# Autodesk Inventor assembly: wheel_screw_joint
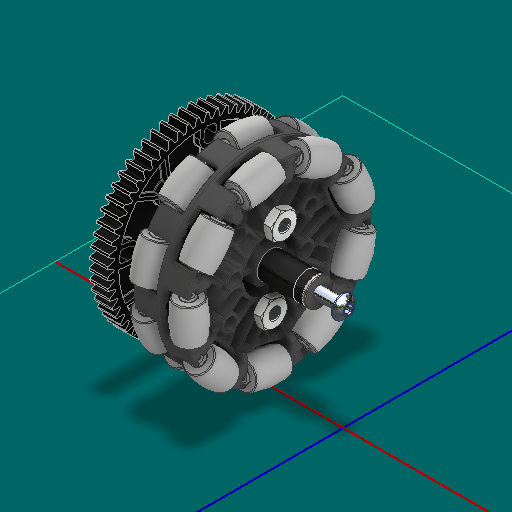
[picture p0: Inventor's stored thumbnail of the model, 512x512]
Saved by Autodesk Inventor 2025 (Build 290162000, 162)
## iProperties
Created: 2024-08-16
Part Number: wheel_screw_joint
Document SubType Name: Assembly
Designer: averey
Author: averey
## Documents named in this file (17)
- C:\Users\avere\vex_robotics_high_stakes\hardware\cad\ATLAS\chassis\drive_pod\wheel_screw_joint.iam
- C:\Users\avere\vex_robotics_high_stakes\hardware\cad\VEX-CAD-Inventor\Structure\Hardware\Screw Steel - Star\SScrew Star Smooth 2.500.ipt
- C:\Users\avere\vex_robotics_high_stakes\hardware\cad\VEX-CAD-Inventor\Structure\Hardware\Screw Steel - Star.ipt
- C:\Users\avere\vex_robotics_high_stakes\hardware\cad\VEX-CAD-Inventor\Motion\Wheels\Omni Wheel\2.75 Omni AS, No Insert.iam
- C:\Users\avere\vex_robotics_high_stakes\hardware\cad\VEX-CAD-Inventor\Motion\Wheels\Omni Wheel.iam
- C:\Users\avere\vex_robotics_high_stakes\hardware\cad\custom_parts\modified_parts\Half Cut HS 60T Gear.ipt
- C:\Users\avere\vex_robotics_high_stakes\hardware\cad\VEX-CAD-Inventor\Motion\Spacers\Spacer Nylon .375 OD\NSpacer .375 OD x .375.ipt
- C:\Users\avere\vex_robotics_high_stakes\hardware\cad\VEX-CAD-Inventor\Motion\Spacers\Spacer Nylon .375 OD.ipt
- C:\Users\avere\vex_robotics_high_stakes\hardware\cad\VEX-CAD-Inventor\Motion\Spacers\Washer Steel\SWasher .375 OD x .015625.ipt
- C:\Users\avere\vex_robotics_high_stakes\hardware\cad\VEX-CAD-Inventor\Motion\Spacers\Washer Steel.ipt
- C:\Users\avere\vex_robotics_high_stakes\hardware\cad\VEX-CAD-Inventor\Motion\Spacers\Washer Steel\SWasher .375 OD x .031250.ipt
- C:\Users\avere\vex_robotics_high_stakes\hardware\cad\VEX-CAD-Inventor\Motion\Spacers\Washer Steel\SWasher .375 OD x .062500.ipt
- C:\Users\avere\vex_robotics_high_stakes\hardware\cad\VEX-CAD-Inventor\Structure\Hardware\Screw Steel - Star\SScrew Star Smooth 1.500.ipt
- C:\Users\avere\vex_robotics_high_stakes\hardware\cad\VEX-CAD-Inventor\Structure\Hardware\Nut Nylon\Nut Nylon - White.ipt
- C:\Users\avere\vex_robotics_high_stakes\hardware\cad\VEX-CAD-Inventor\Structure\Hardware\Nut Nylon.ipt
- C:\Users\avere\vex_robotics_high_stakes\hardware\cad\VEX-CAD-Inventor\Motion\Spacers\Spacer Nylon .375 OD\NSpacer .375 OD x .125.ipt
- C:\Users\avere\vex_robotics_high_stakes\hardware\cad\VEX-CAD-Inventor\Motion\Spacers\Spacer Nylon .375 OD\NSpacer .375 OD x .500.ipt
## Components (19 placed, 11 different names)
1. SScrew Star Smooth 2.500:1 — Mate:1, Mate:2
2. 2.75 Omni AS, No Insert:1 [sub-assembly] — Insert:9, Insert:10, Insert:11, Insert:12, Insert:18
3. Half Cut HS 60T Gear:1 — Mate:3, Insert:13, Insert:14
4. NSpacer .375 OD x .375:1 — Insert:5, Insert:9
5. SWasher .375 OD x .015625:1 — Insert:4
6. SWasher .375 OD x .031250:2 — Insert:3, Insert:4, Mate:3
7. SWasher .375 OD x .062500:3 — Insert:3, Insert:5
8. NSpacer .375 OD x .375:2 — Insert:10
9. SWasher .375 OD x .015625:4
10. SWasher .375 OD x .031250:5
11. SWasher .375 OD x .062500:6
12. SScrew Star Smooth 1.500:2 — Insert:14
13. SScrew Star Smooth 1.500:3 — Insert:13
14. Nut Nylon - White:1 — Insert:11
15. Nut Nylon - White:2 — Insert:12
16. NSpacer .375 OD x .125:3 — Insert:16, Insert:17
17. NSpacer .375 OD x .500:4 — Insert:16, Insert:18
18. SWasher .375 OD x .015625:7 — Insert:15
19. SWasher .375 OD x .031250:8 — Insert:15, Insert:17
## Relationships (21: Insert 18, Mate 3)
- [Insert] (25.4 mm): SScrew Star Smooth 2.500:1 ↔ 2.75 Omni AS, No Insert:1
- [Insert] (9.1281 mm): 2.75 Omni AS, No Insert:1 ↔ Half Cut HS 60T Gear:1
- Mate:1: SScrew Star Smooth 2.500:1
- Mate:2: SScrew Star Smooth 2.500:1
- Insert:3: SWasher .375 OD x .031250:2 ↔ SWasher .375 OD x .062500:3
- Insert:4: SWasher .375 OD x .015625:1 ↔ SWasher .375 OD x .031250:2
- Insert:5: NSpacer .375 OD x .375:1 ↔ SWasher .375 OD x .062500:3
- [Insert]: SWasher .375 OD x .031250:5 ↔ SWasher .375 OD x .062500:6
- [Insert]: SWasher .375 OD x .015625:4 ↔ SWasher .375 OD x .031250:5
- [Insert]: NSpacer .375 OD x .375:2 ↔ SWasher .375 OD x .062500:6
- Insert:9: 2.75 Omni AS, No Insert:1 ↔ NSpacer .375 OD x .375:1
- Insert:10: 2.75 Omni AS, No Insert:1 ↔ NSpacer .375 OD x .375:2
- Mate:3: Half Cut HS 60T Gear:1 ↔ SWasher .375 OD x .031250:2
- Insert:11: 2.75 Omni AS, No Insert:1 ↔ Nut Nylon - White:1
- Insert:12: 2.75 Omni AS, No Insert:1 ↔ Nut Nylon - White:2
- Insert:13: Half Cut HS 60T Gear:1 ↔ SScrew Star Smooth 1.500:3
- Insert:14: Half Cut HS 60T Gear:1 ↔ SScrew Star Smooth 1.500:2
- Insert:15: SWasher .375 OD x .015625:7 ↔ SWasher .375 OD x .031250:8
- Insert:16: NSpacer .375 OD x .125:3 ↔ NSpacer .375 OD x .500:4
- Insert:17: NSpacer .375 OD x .125:3 ↔ SWasher .375 OD x .031250:8
- Insert:18: 2.75 Omni AS, No Insert:1 ↔ NSpacer .375 OD x .500:4
## Named parameters: d7_d4 = 0 mm, d8_d5 = 0 mm, d9_d6 = 0 mm
